# Autodesk Inventor assembly: Assembly
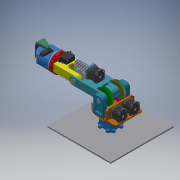
[picture p0: Inventor's stored thumbnail of the model, 180x180]
Saved by Autodesk Inventor 2019 (Build 230136000, 136)
## iProperties
Created: 2019-12-22
Part Number: Assembly
Material: Типовые
Document SubType Name: Assembly
Designer: Петров Иван
Author: Петров Иван
## Documents named in this file (7)
- E:\IVAN\Ivan_desktop\GitHub\Arm_manip\hardware\МД.001.000 - Манипулятор.iam
- E:\IVAN\Ivan_desktop\GitHub\Arm_manip\hardware\МД.001.001 - Основание.ipt
- E:\IVAN\Ivan_desktop\GitHub\Arm_manip\hardware\МД.001.100 - База поворотного стола.iam
- E:\IVAN\Ivan_desktop\GitHub\Arm_manip\hardware\МД.001.200 - Редуктор планетарный.iam
- E:\IVAN\Ivan_desktop\GitHub\Arm_manip\hardware\МД.001.300 - Звено 1.iam
- E:\IVAN\Ivan_desktop\GitHub\Arm_manip\hardware\МД.001.600 - Звено 2.iam
- E:\IVAN\Ivan_desktop\GitHub\Arm_manip\hardware\МД.001.800 - Звено 3.iam
## Components (6 placed, 6 different names)
1. МД.001.001 - Основание:1 — Совмещение:1, Совмещение:2, Совмещение:3, Замок звена 1, Замок горизонтального поворота
2. МД.001.100 - База поворотного стола:1 [sub-assembly] — Совмещение:1, Совмещение:2, Совмещение:3, Совмещение:16, Совмещение:17, Совмещение:18
3. МД.001.300 - Звено 1:1 [sub-assembly] — Совмещение:10, Заподлицо:1, Совмещение:11, Совмещение:12, Замок звена 2, Замок звена 1, Совмещение:19, Совмещение:20, Совмещение:21, Замок горизонтального поворота
4. МД.001.600 - Звено 2:1 [sub-assembly] — Совмещение:10, Заподлицо:1, Совмещение:11, Совмещение:12, Замок звена 2, Совмещение:13, Совмещение:14, Совмещение:15, Замок звена 3
5. МД.001.800 - Звено 3:1 [sub-assembly] — Совмещение:13, Совмещение:14, Совмещение:15, Замок звена 3
6. МД.001.200 - Редуктор планетарный:1 [sub-assembly] — Совмещение:16, Совмещение:17, Совмещение:18, Совмещение:19, Совмещение:20, Совмещение:21
## Relationships (20: Mate 15, Angle 4, Flush 1)
- Совмещение:1 [Mate]: МД.001.001 - Основание:1 ↔ МД.001.100 - База поворотного стола:1
- Совмещение:2 [Mate]: МД.001.001 - Основание:1 ↔ МД.001.100 - База поворотного стола:1
- Совмещение:3 [Mate]: МД.001.001 - Основание:1 ↔ МД.001.100 - База поворотного стола:1
- Совмещение:10 [Mate]: МД.001.300 - Звено 1:1 ↔ МД.001.600 - Звено 2:1
- Заподлицо:1 [Flush]: МД.001.300 - Звено 1:1 ↔ МД.001.600 - Звено 2:1
- Совмещение:11 [Mate]: МД.001.300 - Звено 1:1 ↔ МД.001.600 - Звено 2:1
- Совмещение:12 [Mate]: МД.001.300 - Звено 1:1 ↔ МД.001.600 - Звено 2:1
- Замок звена 2 [Angle] (0 deg): МД.001.300 - Звено 1:1 ↔ МД.001.600 - Звено 2:1
- Совмещение:13 [Mate]: МД.001.600 - Звено 2:1 ↔ МД.001.800 - Звено 3:1
- Совмещение:14 [Mate]: МД.001.600 - Звено 2:1 ↔ МД.001.800 - Звено 3:1
- Совмещение:15 [Mate]: МД.001.600 - Звено 2:1 ↔ МД.001.800 - Звено 3:1
- Замок звена 1 [Angle] (0 deg): МД.001.001 - Основание:1 ↔ МД.001.300 - Звено 1:1
- Совмещение:16 [Mate]: МД.001.100 - База поворотного стола:1 ↔ МД.001.200 - Редуктор планетарный:1
- Совмещение:17 [Mate]: МД.001.100 - База поворотного стола:1 ↔ МД.001.200 - Редуктор планетарный:1
- Совмещение:18 [Mate]: МД.001.100 - База поворотного стола:1 ↔ МД.001.200 - Редуктор планетарный:1
- Совмещение:19 [Mate]: МД.001.300 - Звено 1:1 ↔ МД.001.200 - Редуктор планетарный:1
- Совмещение:20 [Mate]: МД.001.300 - Звено 1:1 ↔ МД.001.200 - Редуктор планетарный:1
- Совмещение:21 [Mate]: МД.001.300 - Звено 1:1 ↔ МД.001.200 - Редуктор планетарный:1
- Замок горизонтального поворота [Angle] (0 deg): МД.001.001 - Основание:1 ↔ МД.001.300 - Звено 1:1
- Замок звена 3 [Angle] (0 deg): МД.001.600 - Звено 2:1 ↔ МД.001.800 - Звено 3:1
